# Autodesk Inventor assembly: real joint assemly
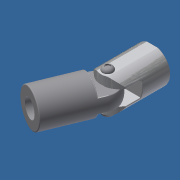
[picture p0: Inventor's stored thumbnail of the model, 180x180]
Saved by Autodesk Inventor 2018 (Build 220112000, 112)
## iProperties
Created: 2018-04-06
Part Number: real joint assemly
Document SubType Name: Assembly
Designer: 232963
Author: 232963
## Documents named in this file (5)
- P:\IED\SchoolCAD\Design Challenge\real joint assemly.iam
- P:\IED\SchoolCAD\Design Challenge\joint 2.ipt
- P:\IED\SchoolCAD\Design Challenge\joint 4.ipt
- P:\IED\SchoolCAD\Design Challenge\Part3.ipt
- P:\IED\SchoolCAD\Design Challenge\Screw.ipt
## Components (4 placed, 4 different names)
1. joint 2:1 — Insert:1, Insert:2, Insert:3, Insert:4, Insert:5
2. joint 4:1 — Insert:1, Insert:2, Insert:5
3. Part3:1 — Insert:3
4. Screw:1 — Insert:4
## Relationships (5: Insert 5)
- Insert:1: joint 2:1 ↔ joint 4:1
- Insert:2 (0.508 mm): joint 2:1 ↔ joint 4:1
- Insert:3: joint 2:1 ↔ Part3:1
- Insert:4: joint 2:1 ↔ Screw:1
- Insert:5: joint 2:1 ↔ joint 4:1
